# Autodesk Inventor assembly: Potential gripper3
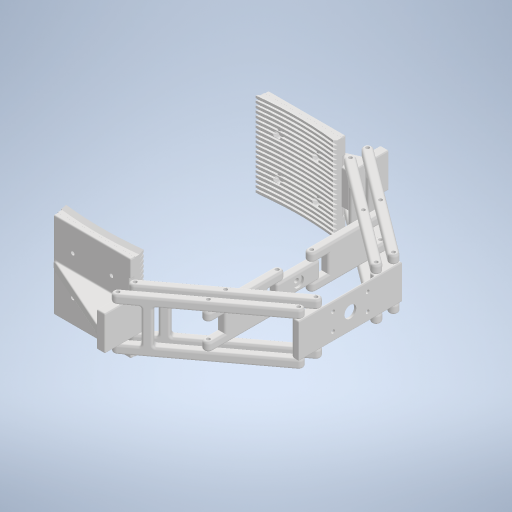
[picture p0: Inventor's stored thumbnail of the model, 512x512]
Saved by Autodesk Inventor 2023 (Build 270158000, 158)
## iProperties
Created: 2023-02-07
Part Number: Potential gripper3
Document SubType Name: Assembly
Designer: Gabriel - T3 CAD
Author: Gabriel - T3 CAD
## Documents named in this file (12)
- C:\Users\Gabriel - T3 CAD\Documents\GitHub\T3-CAD\Current Season CAD\Swerve-DriveTrain-V2.1 (LongBot)\Potential new gripper\Potential gripper3.iam
- C:\Users\Gabriel - T3 CAD\Documents\GitHub\T3-CAD\Current Season CAD\Swerve-DriveTrain-V2.1 (LongBot)\Potential new gripper\Finger.ipt
- C:\Users\Gabriel - T3 CAD\Documents\GitHub\T3-CAD\Current Season CAD\Swerve-DriveTrain-V2.1 (LongBot)\Potential new gripper\inner swing.ipt
- C:\Users\Gabriel - T3 CAD\Documents\GitHub\T3-CAD\Current Season CAD\Swerve-DriveTrain-V2.1 (LongBot)\Potential new gripper\piston connection.ipt
- C:\Users\Gabriel - T3 CAD\Documents\GitHub\T3-CAD\Current Season CAD\Swerve-DriveTrain-V2.1 (LongBot)\Potential new gripper\swing pusher.ipt
- C:\Users\Gabriel - T3 CAD\Documents\GitHub\T3-CAD\Current Season CAD\Swerve-DriveTrain-V2.1 (LongBot)\Potential new gripper\Connector plate.ipt
- C:\Users\Gabriel - T3 CAD\Documents\GitHub\T3-CAD\Stock\ThriftyBot-Elevator\Configurable Thrifty Elevator_Simplify_2.ipt
- C:\Users\Gabriel - T3 CAD\Documents\GitHub\T3-CAD\Current Season CAD\Swerve-DriveTrain-V2.1 (LongBot)\Potential new gripper\inner swing_MIR.ipt
- C:\Users\Gabriel - T3 CAD\Documents\GitHub\T3-CAD\Current Season CAD\Swerve-DriveTrain-V2.1 (LongBot)\Potential new gripper\swing pusher_MIR.ipt
- C:\Users\Gabriel - T3 CAD\Documents\GitHub\T3-CAD\Current Season CAD\Swerve-DriveTrain-V2.1 (LongBot)\Potential new gripper\Gripper plate v2.ipt
- C:\Users\Gabriel - T3 CAD\Documents\GitHub\T3-CAD\Current Season CAD\Swerve-DriveTrain-V2.1 (LongBot)\Potential new gripper\Finger_MIR1.ipt
- C:\Users\Gabriel - T3 CAD\Documents\GitHub\T3-CAD\Current Season CAD\Swerve-DriveTrain-V2.1 (LongBot)\Potential new gripper\Gripper plate v2_MIR.ipt
## Components (13 placed, 11 different names)
1. Finger:1 — Rotational:37, Rotational:38, Rotational:44, Rotational:46
2. inner swing:2 — Rotational:33, Rotational:37, Rotational:43
3. piston connection:1 — Cylindrical:1, Rotational:41, Rotational:42, Angle:2
4. swing pusher:1 — Rotational:42, Rotational:43
5. Connector plate:2 — Rotational:7, Angle:1, Cylindrical:1, Rotational:33, Rotational:34, Rotational:35, Rotational:36
6. Configurable Thrifty Elevator_Simplify_2:1 — Rotational:7, Angle:1
7. inner swing_MIR:1 — Rotational:32, Rotational:34, Rotational:49
8. swing pusher_MIR:1 — Rotational:32, Rotational:41, Angle:2
9. inner swing:3 — Rotational:35, Rotational:38
10. inner swing_MIR:2 — Rotational:36, Rotational:50
11. Gripper plate v2:1 — Rotational:44, Rotational:46
12. Finger_MIR1:1 — Rotational:47, Rotational:48, Rotational:49, Rotational:50
13. Gripper plate v2_MIR:1 — Rotational:47, Rotational:48
## Relationships (20: RevoluteJoint 17, Angle 2, CylindricalJoint 1)
- Rotational:7 [RevoluteJoint]: Connector plate:2 ↔ Configurable Thrifty Elevator_Simplify_2:1
- Angle:1 (90 deg): Connector plate:2 ↔ Configurable Thrifty Elevator_Simplify_2:1
- Cylindrical:1: piston connection:1 ↔ Connector plate:2
- Rotational:32 [RevoluteJoint]: inner swing_MIR:1 ↔ swing pusher_MIR:1
- Rotational:33 [RevoluteJoint]: inner swing:2 ↔ Connector plate:2
- Rotational:34 [RevoluteJoint]: Connector plate:2 ↔ inner swing_MIR:1
- Rotational:35 [RevoluteJoint]: Connector plate:2 ↔ inner swing:3
- Rotational:36 [RevoluteJoint]: Connector plate:2 ↔ inner swing_MIR:2
- Rotational:37 [RevoluteJoint]: Finger:1 ↔ inner swing:2
- Rotational:38 [RevoluteJoint]: Finger:1 ↔ inner swing:3
- Rotational:41 [RevoluteJoint]: piston connection:1 ↔ swing pusher_MIR:1
- Rotational:42 [RevoluteJoint]: piston connection:1 ↔ swing pusher:1
- Rotational:43 [RevoluteJoint]: inner swing:2 ↔ swing pusher:1
- Angle:2 (0 deg): piston connection:1 ↔ swing pusher_MIR:1
- Rotational:44 [RevoluteJoint]: Finger:1 ↔ Gripper plate v2:1
- Rotational:46 [RevoluteJoint]: Finger:1 ↔ Gripper plate v2:1
- Rotational:47 [RevoluteJoint]: Finger_MIR1:1 ↔ Gripper plate v2_MIR:1
- Rotational:48 [RevoluteJoint]: Finger_MIR1:1 ↔ Gripper plate v2_MIR:1
- Rotational:49 [RevoluteJoint]: inner swing_MIR:1 ↔ Finger_MIR1:1
- Rotational:50 [RevoluteJoint]: inner swing_MIR:2 ↔ Finger_MIR1:1
